# Autodesk Inventor assembly: resevoir_mount
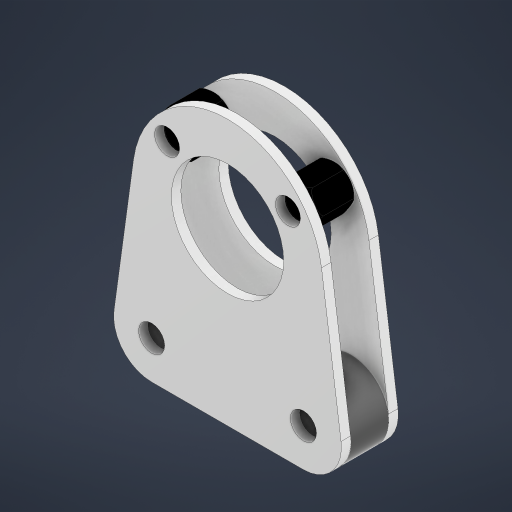
[picture p0: Inventor's stored thumbnail of the model, 512x512]
Saved by Autodesk Inventor 2024 (Build 280153000, 153)
## iProperties
Created: 2024-01-16
Part Number: resevoir_mount
Document SubType Name: Assembly
Designer: avere
Author: avere
## Documents named in this file (6)
- C:\Users\avere\Documents\rbp_cad\zoomba_v0.3\chassis\resevoir_mount.iam
- C:\Users\avere\Documents\rbp_cad\zoomba_v0.3\chassis\custom_parts\resevoir_mount.ipt
- C:\Users\avere\Documents\rbp_cad\VEX-CAD-Inventor-1.41\Motion\Spacers\Spacer Nylon .500 OD\NSpacer Black .500 OD x .250.ipt
- C:\Users\avere\Documents\rbp_cad\VEX-CAD-Inventor-1.41\Motion\Spacers\Spacer Nylon .500 OD.ipt
- C:\Users\avere\Documents\rbp_cad\VEX-CAD-Inventor-1.41\Structure\Standoff\Standoff .25.ipt
- C:\Users\avere\Documents\rbp_cad\VEX-CAD-Inventor-1.41\Structure\Standoff.ipt
## Components (6 placed, 3 different names)
1. resevoir_mount:1 — Insert:1, Mate:1
2. resevoir_mount:2 — Insert:1, Mate:1, Insert:2, Insert:3, Insert:4, Insert:5
3. NSpacer Black .500 OD x .250:1 — Insert:2
4. NSpacer Black .500 OD x .250:2 — Insert:3
5. Standoff .25:1 — Insert:4
6. Standoff .25:2 — Insert:5
## Relationships (6: Insert 5, Mate 1)
- Insert:1 (6.35 mm): resevoir_mount:1 ↔ resevoir_mount:2
- Mate:1: resevoir_mount:1 ↔ resevoir_mount:2
- Insert:2: resevoir_mount:2 ↔ NSpacer Black .500 OD x .250:1
- Insert:3: resevoir_mount:2 ↔ NSpacer Black .500 OD x .250:2
- Insert:4: resevoir_mount:2 ↔ Standoff .25:1
- Insert:5: resevoir_mount:2 ↔ Standoff .25:2
